# Autodesk Inventor assembly: enormous-gear
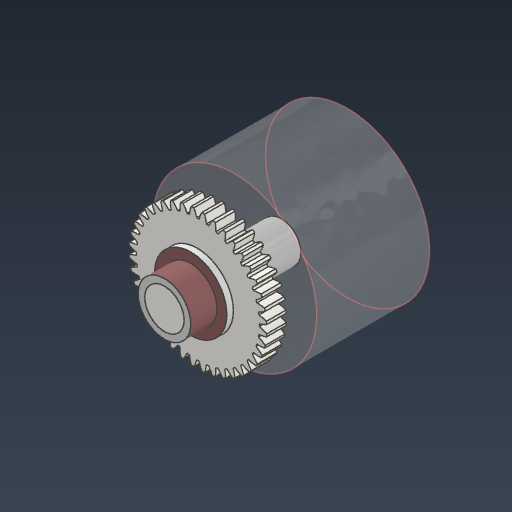
[picture p0: Inventor's stored thumbnail of the model, 512x512]
Saved by Autodesk Inventor 2023 (Build 270158000, 158)
## iProperties
Created: 2025-04-01
Part Number: enormous-gear
Document SubType Name: Assembly
Designer: szymo
Author: szymo
## Documents named in this file (5)
- D:\tech\robotyka\robots\evangelion\inventor-project\enormous-gear-short.iam
- D:\tech\robotyka\robots\evangelion\inventor-project\Gears\Design Accelerator\Przekładnia walcowa24.ipt
- D:\tech\robotyka\robots\evangelion\inventor-project\wheel.ipt
- D:\tech\robotyka\robots\evangelion\inventor-project\bearing SF-1F-6mm.ipt
- D:\tech\robotyka\robots\evangelion\inventor-project\bearing SF-1F-very_short.ipt
## Components (4 placed, 4 different names)
1. Przekładnia walcowa2:1 — Mate:3, Mate:4, Mate:5, Mate:6, Mate:7, Mate:8
2. wheel:1 — Mate:3, Mate:4
3. bearing SF-1F-6mm:1 — Mate:5, Mate:6
4. bearing SF-1F-very_short:1 — Mate:7, Mate:8
## Relationships (6: Mate 6)
- Mate:3: Przekładnia walcowa2:1 ↔ wheel:1
- Mate:4 (2.6 mm): Przekładnia walcowa2:1 ↔ wheel:1
- Mate:5 (0.1 mm): Przekładnia walcowa2:1 ↔ bearing SF-1F-6mm:1
- Mate:6: Przekładnia walcowa2:1 ↔ bearing SF-1F-6mm:1
- Mate:7 (0.1 mm): Przekładnia walcowa2:1 ↔ bearing SF-1F-very_short:1
- Mate:8: Przekładnia walcowa2:1 ↔ bearing SF-1F-very_short:1
